# Autodesk Inventor assembly: Assembly
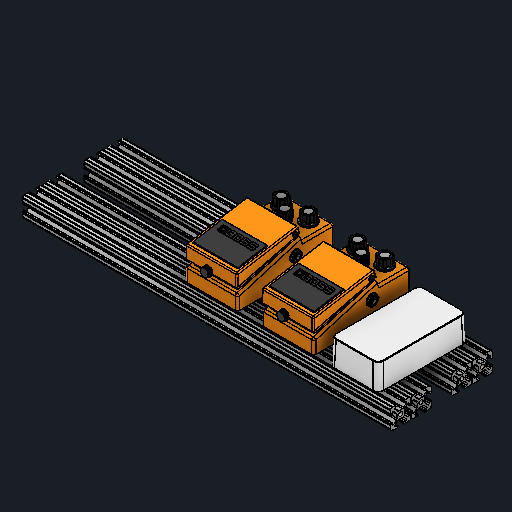
[picture p0: Inventor's stored thumbnail of the model, 512x512]
Saved by Autodesk Inventor 2026.2 (Build 302298000, 298)
## iProperties
Created: 2026-05-18
Part Number: Assembly
Document SubType Name: Assembly
Designer: JoshuaEah
Author: JoshuaEah
## Documents named in this file (5)
- C:\Users\JoshuaEah\Documents\GitHub\Designed-Trinkets\Guitar\Modular Pedalboard\Assembly.iam
- C:\Users\JoshuaEah\Documents\GitHub\Designed-Trinkets\Guitar\Modular Pedalboard\1x1 Alu Extrusion.ipt
- 1x1" Alu Extrusion.ipt
- C:\Users\JoshuaEah\Documents\GitHub\Designed-Trinkets\Guitar\Modular Pedalboard\Pedals\Compressor.ipt
- C:\Users\JoshuaEah\Documents\GitHub\Designed-Trinkets\Guitar\Modular Pedalboard\Pedals\Boss Pedal\Boss_Assembly.iam
## Components (7 placed, 3 different names)
1. 1x1 Alu Extrusion:1 — Flush:1, Flush:2, Flush:3, Flush:4, Mate:12, Mate:15, Mate:16, Angle:1, Mate:17, Angle:2
2. 1x1 Alu Extrusion:2 — Flush:1, Flush:4, Flush:5, Mate:12, Mate:13
3. 1x1 Alu Extrusion:3 — Flush:2, Flush:5, Flush:6, Mate:13, Mate:14
4. 1x1 Alu Extrusion:4 — Flush:3, Flush:6, Mate:14
5. Compressor:1 — Mate:15
6. Boss_Assembly:1 [sub-assembly] — Mate:16, Angle:1
7. Boss_Assembly:2 [sub-assembly] — Mate:17, Angle:2
## Relationships (14: Flush 6, Mate 6, Angle 2)
- Flush:1: 1x1 Alu Extrusion:1 ↔ 1x1 Alu Extrusion:2
- Flush:2: 1x1 Alu Extrusion:1 ↔ 1x1 Alu Extrusion:3
- Flush:3: 1x1 Alu Extrusion:1 ↔ 1x1 Alu Extrusion:4
- Flush:4: 1x1 Alu Extrusion:1 ↔ 1x1 Alu Extrusion:2
- Flush:5: 1x1 Alu Extrusion:2 ↔ 1x1 Alu Extrusion:3
- Flush:6: 1x1 Alu Extrusion:3 ↔ 1x1 Alu Extrusion:4
- Mate:12: 1x1 Alu Extrusion:1 ↔ 1x1 Alu Extrusion:2
- Mate:13 (25.4 mm): 1x1 Alu Extrusion:2 ↔ 1x1 Alu Extrusion:3
- Mate:14: 1x1 Alu Extrusion:3 ↔ 1x1 Alu Extrusion:4
- Mate:15: 1x1 Alu Extrusion:1 ↔ Compressor:1
- Mate:16: 1x1 Alu Extrusion:1 ↔ Boss_Assembly:1
- Angle:1 (0 deg): 1x1 Alu Extrusion:1 ↔ Boss_Assembly:1
- Mate:17: 1x1 Alu Extrusion:1 ↔ Boss_Assembly:2
- Angle:2 (0 deg): 1x1 Alu Extrusion:1 ↔ Boss_Assembly:2
